# Autodesk Inventor assembly: A2017_T5_03
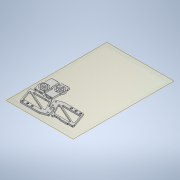
[picture p0: Inventor's stored thumbnail of the model, 180x180]
Saved by Autodesk Inventor 2020 (Build 240168000, 168)
## iProperties
Created: 2021-08-27
Part Number: A2017_T5_03
Document SubType Name: Assembly
Designer: Masato
Author: Masato
## Documents named in this file (4)
- C:\Users\naoki\Documents\Inventor\CitBrains\git_clone\OpenPlatform4_0\A2017_T5_03\OpenPlatform_ver3_0\cam\A2017_T5_03.iam
- C:\Users\naoki\Documents\Inventor\CitBrains\git_clone\OpenPlatform4_0\A2017_T5_03\OpenPlatform_ver3_0\cam\Disposable_Board.ipt
- C:\Users\naoki\Documents\Inventor\CitBrains\git_clone\OpenPlatform4_0\A2017_T5_03\OpenPlatform_ver3_0\LowerBody\Leg_joit\Leg_joint_yaw_frame.ipt
- C:\Users\naoki\Documents\Inventor\CitBrains\git_clone\OpenPlatform4_0\A2017_T5_03\OpenPlatform_ver3_0\UpperBody\Trunk\Trunk_lower_flank_frame.ipt
## Components (5 placed, 3 different names)
1. Disposable_Board:1 — メイト:2, メイト:1, フラッシュ:1, フラッシュ:2, メイト:4, メイト:5, メイト:6, メイト:7, フラッシュ:3, フラッシュ:4, 正接:1
2. Leg_joint_yaw_frame:1 — メイト:4, 正接:1, メイト:10, 正接:2
3. Leg_joint_yaw_frame:2 — メイト:5, メイト:11, 正接:2
4. Trunk_lower_flank_frame:1 — メイト:7, フラッシュ:3, フラッシュ:4, メイト:8, メイト:9, メイト:10, メイト:11
5. Trunk_lower_flank_frame:2 — メイト:6, メイト:8, メイト:9
## Relationships (16: Mate 10, Flush 4, Tangent 2)
- メイト:2 [Mate]: Disposable_Board:1
- メイト:1 [Mate]: Disposable_Board:1
- フラッシュ:1 [Flush]: Disposable_Board:1
- フラッシュ:2 [Flush]: Disposable_Board:1
- メイト:4 [Mate]: Disposable_Board:1 ↔ Leg_joint_yaw_frame:1
- メイト:5 [Mate]: Disposable_Board:1 ↔ Leg_joint_yaw_frame:2
- メイト:6 [Mate]: Disposable_Board:1 ↔ Trunk_lower_flank_frame:2
- メイト:7 [Mate]: Disposable_Board:1 ↔ Trunk_lower_flank_frame:1
- フラッシュ:3 [Flush] (2 mm): Disposable_Board:1 ↔ Trunk_lower_flank_frame:1
- フラッシュ:4 [Flush] (2 mm): Disposable_Board:1 ↔ Trunk_lower_flank_frame:1
- メイト:8 [Mate] (2.5 mm): Trunk_lower_flank_frame:1 ↔ Trunk_lower_flank_frame:2
- メイト:9 [Mate] (2.5 mm): Trunk_lower_flank_frame:1 ↔ Trunk_lower_flank_frame:2
- 正接:1 [Tangent] (2 mm): Disposable_Board:1 ↔ Leg_joint_yaw_frame:1
- メイト:10 [Mate] (2.5 mm): Leg_joint_yaw_frame:1 ↔ Trunk_lower_flank_frame:1
- メイト:11 [Mate] (2.5 mm): Leg_joint_yaw_frame:2 ↔ Trunk_lower_flank_frame:1
- 正接:2 [Tangent] (2.5 mm): Leg_joint_yaw_frame:1 ↔ Leg_joint_yaw_frame:2
